# Autodesk Inventor assembly: NT_NCS002_003_P01
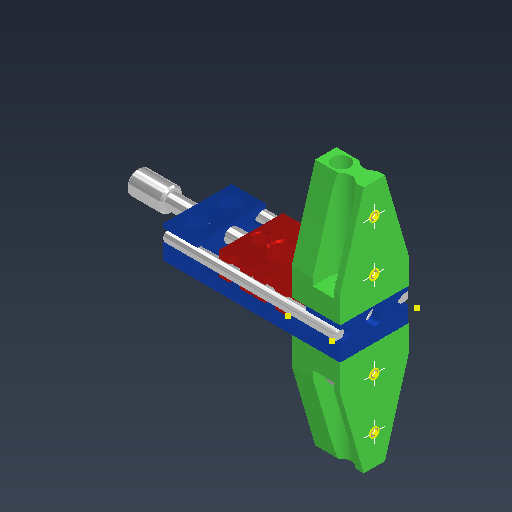
[picture p0: Inventor's stored thumbnail of the model, 512x512]
Saved by Autodesk Inventor 2026.2 (Build 302298010, 298A)
## iProperties
Manager: Gozzi
Company: IIT
Created: 2026-03-26
Part Number: NT_NCS002_003_P01
Document SubType Name: Assembly
Designer: Fabio Ricci
Mass: 6.15858 g
Surface Area: 38.7489 cm^2
Volume: 2.14557 cm^3
Density: 2.87037 g/cm^3
Description: Probe holder edmund coupled
Title: Ephys_probe_holder
Author: Fabio Ricci
## Documents named in this file (7)
- C:\Users\faricci\OneDrive - Fondazione Istituto Italiano Tecnologia\Desktop\NT_NCS002_003_A_01.iam
- C:\Users\faricci\OneDrive - Fondazione Istituto Italiano Tecnologia\Desktop\NT_NCS002_003_P_01.ipt
- C:\Users\faricci\OneDrive - Fondazione Istituto Italiano Tecnologia\Desktop\NT_NCS002_003_P_02.ipt
- C:\Users\faricci\OneDrive - Fondazione Istituto Italiano Tecnologia\Desktop\#56-419.ipt
- C:\Users\faricci\OneDrive - Fondazione Istituto Italiano Tecnologia\Desktop\Probe_Holder\Design Accelerator\Bolted Connection2.iam
- C:\Users\faricci\OneDrive - Fondazione Istituto Italiano Tecnologia\Desktop\Probe_Holder\Design Accelerator\Bolted Connection3.iam
- C:\Users\faricci\OneDrive - Fondazione Istituto Italiano Tecnologia\Documents\Inventor\Content Center Files\R2026\en-US\ISO 4026\ISO 4026 - M1.6 x 2 - ISO.ipt
## Components (9 placed, 5 different names)
1. Part2 — Rigid:1, Mate:4, Mate:6, Mate:9, Mate:10
2. NT_NCS002_003_P_02:1 — Rigid:2, Mate:3, Mate:5, Mate:7, Mate:8
3. #56-419:1 — Rigid:1, Rigid:2
4. Bolted Connection:1 [sub-assembly] — Mate:5, Mate:6
5. Bolted Connection:2 [sub-assembly] — Mate:3, Mate:4
6. ISO 4026 M1.6 x 2:1 — Mate:7
7. ISO 4026 M1.6 x 2:2 — Mate:8
8. ISO 4026 M1.6 x 2:3 — Mate:9
9. ISO 4026 M1.6 x 2:4 — Mate:10
## Relationships (10: Mate 8, WeldJoint 2)
- Rigid:1 [WeldJoint]: Part2 ↔ #56-419:1
- Rigid:2 [WeldJoint]: NT_NCS002_003_P_02:1 ↔ #56-419:1
- Mate:3: NT_NCS002_003_P_02:1 ↔ Bolted Connection:2
- Mate:4: Part2 ↔ Bolted Connection:2
- Mate:5: NT_NCS002_003_P_02:1 ↔ Bolted Connection:1
- Mate:6: Part2 ↔ Bolted Connection:1
- Mate:7: NT_NCS002_003_P_02:1 ↔ ISO 4026 M1.6 x 2:1
- Mate:8: NT_NCS002_003_P_02:1 ↔ ISO 4026 M1.6 x 2:2
- Mate:9: Part2 ↔ ISO 4026 M1.6 x 2:3
- Mate:10: Part2 ↔ ISO 4026 M1.6 x 2:4
